# Autodesk Inventor assembly: MGN12H_400mm
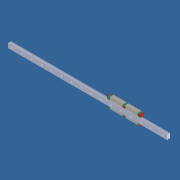
[picture p0: Inventor's stored thumbnail of the model, 180x180]
Saved by Autodesk Inventor 2020 (Build 240168000, 168)
## iProperties
Created: 2020-09-22
Part Number: MGN12H_400mm
Document SubType Name: Assembly
Designer: magnarecta
Title: C:/Users/lvglv/Downloads/MGN12H_400mm.step
## Documents named in this file (3)
- D:\Document\Github\CoreXY_Laser\Model\Parts\Linear_Guide\MGN12H_400mm\MGN12H_400mm.iam
- D:\Document\Github\CoreXY_Laser\Model\Parts\Linear_Guide\MGN12H_400mm\MGN12H, LINEAR GUIDE BLOCK.ipt
- D:\Document\Github\CoreXY_Laser\Model\Parts\Linear_Guide\MGN12H_400mm\MGN12 LINEAR GUIDE RAIL, CONFIGURABLE, 400 mm.ipt
## Components (3 placed, 2 different names)
1. MGN12H, LINEAR GUIDE BLOCK:1 — フラッシュ:1, フラッシュ:2, メイト:1, 角度:1
2. MGN12 LINEAR GUIDE RAIL, CONFIGURABLE, 400 mm:1 — メイト:1, 角度:1
3. MGN12H, LINEAR GUIDE BLOCK:2 — フラッシュ:1, フラッシュ:2
## Relationships (4: Flush 2, Mate 1, Angle 1)
- フラッシュ:1 [Flush]: MGN12H, LINEAR GUIDE BLOCK:1 ↔ MGN12H, LINEAR GUIDE BLOCK:2
- フラッシュ:2 [Flush]: MGN12H, LINEAR GUIDE BLOCK:1 ↔ MGN12H, LINEAR GUIDE BLOCK:2
- メイト:1 [Mate]: MGN12H, LINEAR GUIDE BLOCK:1 ↔ MGN12 LINEAR GUIDE RAIL, CONFIGURABLE, 400 mm:1
- 角度:1 [Angle] (0 deg): MGN12H, LINEAR GUIDE BLOCK:1 ↔ MGN12 LINEAR GUIDE RAIL, CONFIGURABLE, 400 mm:1
